# Autodesk Inventor assembly: McCrea_head_walle
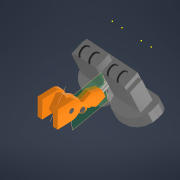
[picture p0: Inventor's stored thumbnail of the model, 180x180]
Saved by Autodesk Inventor 2022 (Build 260153000, 153)
## iProperties
Created: 2022-01-20
Part Number: McCrea_head_walle
Document SubType Name: Assembly
Designer: MatusBarany
Author: MatusBarany
## Documents named in this file (19)
- C:\Users\MatusBarany\Documents\Inventor\wall-e\assembly\McCrea_head_walle.iam
- C:\Users\MatusBarany\Documents\Inventor\wall-e\maxo\McCrea_kabel_walle.ipt
- C:\Users\MatusBarany\Documents\Inventor\wall-e\maxo\McCrea_krk_walle.ipt
- C:\Users\MatusBarany\Documents\Inventor\wall-e\maxo\McCrea_oblucik_walle.ipt
- C:\Users\MatusBarany\Documents\Inventor\wall-e\maxo\McCrea_oko_walle.ipt
- C:\Users\MatusBarany\Documents\Inventor\wall-e\maxo\McCrea_palicka_walle.ipt
- C:\Users\MatusBarany\Documents\Inventor\wall-e\maxo\McCrea_uhco_walle.ipt
- C:\Users\MatusBarany\Documents\Inventor\wall-e\maxo\McCrea_velka_palicka_walle.ipt
- C:\Users\MatusBarany\Documents\Inventor\wall-e\maxo\McCrea_velka_palicka_walle_1.ipt
- C:\Users\MatusBarany\Documents\Inventor\wall-e\maxo\McCrea_velky_krk_walle.ipt
- C:\Users\MatusBarany\Documents\Inventor\wall-e\maxo\McCrea_zadna_cast_oka_walle.ipt
- C:\Users\MatusBarany\Documents\Inventor\wall-e\maxo\McCrea_zadne_oko_walle.ipt
- C:\Users\MatusBarany\Documents\Inventor\wall-e\maxo\McCrea_doska_walle.ipt
- C:\Users\MatusBarany\Documents\Inventor\wall-e\maxo\McCrea_uhco_walle_MIR2.ipt
- C:\Users\MatusBarany\Documents\Inventor\wall-e\maxo\McCrea_zadna_cast_oka_walle_MIR2.ipt
- C:\Users\MatusBarany\Documents\Inventor\wall-e\maxo\McCrea_kabel_walle_MIR.ipt
- C:\Users\MatusBarany\Documents\Inventor\wall-e\maxo\McCrea_oko_walle_MIR2.ipt
- C:\Users\MatusBarany\Documents\Inventor\wall-e\maxo\McCrea_velka_palicka_walle_MIR2.ipt
- C:\Users\MatusBarany\Documents\Inventor\wall-e\maxo\McCrea_zadne_oko_walle_MIR2.ipt
## Components (22 placed, 18 different names)
1. McCrea_krk_walle:1 — Rotational:6, Rotational:8, Insert:2
2. McCrea_oblucik_walle:1 — Rotational:5, Rotational:6, Flush:8
3. McCrea_palicka_walle:1 — Rotational:7
4. McCrea_uhco_walle:1 — Mate:2, Flush:1, Mate:14
5. McCrea_zadna_cast_oka_walle:1 — Rigid:3, Mate:1, Flush:3, Mate:13, Mate:14
6. McCrea_kabel_walle:2 — Mate:3, Mate:15, Mate:16
7. McCrea_oblucik_walle:2 — Rotational:7, Rotational:8, Flush:8
8. McCrea_oko_walle:2 — Rigid:3, Cylindrical:1, Flush:4
9. McCrea_palicka_walle:2 — Rotational:5
10. McCrea_velka_palicka_walle:2 — Cylindrical:1, Flush:4
11. McCrea_velka_palicka_walle_1:2 — Rotational:4, Insert:1
12. McCrea_velky_krk_walle:2 — Insert:1, Flush:2, Insert:2
13. McCrea_zadne_oko_walle:2 — Mate:1, Mate:2, Flush:1, Mate:3, Mate:4, Flush:3, Mate:13, Mate:15, Mate:16, Mate:17, Mate:18, Mate:19, Mate:20, Mate:21
14. McCrea_kabel_walle:3 — Mate:4, Mate:17, Mate:18
15. McCrea_doska_walle:1 — Rotational:4, Mate:19, Mate:20, Mate:21, Flush:9
16. McCrea_uhco_walle_MIR2:1 — Mate:22, Flush:12, Mate:27
17. McCrea_zadna_cast_oka_walle_MIR2:1 — Mate:22, Mate:25, Flush:11, Mate:28, Rigid:4
18. McCrea_kabel_walle_MIR:1 — Mate:23, Mate:24, Mate:26
19. McCrea_oko_walle_MIR2:1 — Flush:10, Rigid:4, Cylindrical:2
20. McCrea_velka_palicka_walle_MIR2:1 — Flush:10, Cylindrical:2
21. McCrea_zadne_oko_walle_MIR2:1 — Mate:23, Mate:24, Mate:25, Flush:11, Mate:26, Flush:12, Mate:27, Mate:28, Mate:29, Mate:30, Mate:31
22. McCrea_kabel_walle_MIR:2 — Mate:29, Mate:30, Mate:31
## Relationships (43: Mate 23, Flush 9, RevoluteJoint 5, WeldJoint 2, Insert 2, CylindricalJoint 2)
- Rigid:3 [WeldJoint]: McCrea_zadna_cast_oka_walle:1 ↔ McCrea_oko_walle:2
- Mate:1: McCrea_zadna_cast_oka_walle:1 ↔ McCrea_zadne_oko_walle:2
- Mate:2: McCrea_uhco_walle:1 ↔ McCrea_zadne_oko_walle:2
- Flush:1: McCrea_uhco_walle:1 ↔ McCrea_zadne_oko_walle:2
- Mate:3: McCrea_kabel_walle:2 ↔ McCrea_zadne_oko_walle:2
- Mate:4: McCrea_zadne_oko_walle:2 ↔ McCrea_kabel_walle:3
- Rotational:4 [RevoluteJoint]: McCrea_velka_palicka_walle_1:2 ↔ McCrea_doska_walle:1
- Insert:1: McCrea_velka_palicka_walle_1:2 ↔ McCrea_velky_krk_walle:2
- Flush:2 (-3.5 mm): McCrea_velky_krk_walle:2
- Flush:3: McCrea_zadna_cast_oka_walle:1 ↔ McCrea_zadne_oko_walle:2
- Cylindrical:1: McCrea_oko_walle:2 ↔ McCrea_velka_palicka_walle:2
- Flush:4: McCrea_oko_walle:2 ↔ McCrea_velka_palicka_walle:2
- Rotational:5 [RevoluteJoint]: McCrea_oblucik_walle:1 ↔ McCrea_palicka_walle:2
- Rotational:6 [RevoluteJoint]: McCrea_krk_walle:1 ↔ McCrea_oblucik_walle:1
- Rotational:7 [RevoluteJoint]: McCrea_palicka_walle:1 ↔ McCrea_oblucik_walle:2
- Rotational:8 [RevoluteJoint]: McCrea_krk_walle:1 ↔ McCrea_oblucik_walle:2
- Flush:8: McCrea_oblucik_walle:1 ↔ McCrea_oblucik_walle:2
- Mate:13: McCrea_zadna_cast_oka_walle:1 ↔ McCrea_zadne_oko_walle:2
- Mate:14: McCrea_uhco_walle:1 ↔ McCrea_zadna_cast_oka_walle:1
- Mate:15: McCrea_kabel_walle:2 ↔ McCrea_zadne_oko_walle:2
- Mate:16: McCrea_kabel_walle:2 ↔ McCrea_zadne_oko_walle:2
- Mate:17: McCrea_zadne_oko_walle:2 ↔ McCrea_kabel_walle:3
- Mate:18: McCrea_zadne_oko_walle:2 ↔ McCrea_kabel_walle:3
- Mate:19: McCrea_zadne_oko_walle:2 ↔ McCrea_doska_walle:1
- Mate:20: McCrea_zadne_oko_walle:2 ↔ McCrea_doska_walle:1
- Mate:21: McCrea_zadne_oko_walle:2 ↔ McCrea_doska_walle:1
- Insert:2: McCrea_krk_walle:1 ↔ McCrea_velky_krk_walle:2
- Flush:9 (-4 mm): McCrea_doska_walle:1
- Mate:22: McCrea_uhco_walle_MIR2:1 ↔ McCrea_zadna_cast_oka_walle_MIR2:1
- Flush:10: McCrea_oko_walle_MIR2:1 ↔ McCrea_velka_palicka_walle_MIR2:1
- Mate:23: McCrea_kabel_walle_MIR:1 ↔ McCrea_zadne_oko_walle_MIR2:1
- Mate:24: McCrea_kabel_walle_MIR:1 ↔ McCrea_zadne_oko_walle_MIR2:1
- Mate:25: McCrea_zadna_cast_oka_walle_MIR2:1 ↔ McCrea_zadne_oko_walle_MIR2:1
- Flush:11: McCrea_zadna_cast_oka_walle_MIR2:1 ↔ McCrea_zadne_oko_walle_MIR2:1
- Mate:26: McCrea_kabel_walle_MIR:1 ↔ McCrea_zadne_oko_walle_MIR2:1
- Flush:12: McCrea_uhco_walle_MIR2:1 ↔ McCrea_zadne_oko_walle_MIR2:1
- Mate:27: McCrea_uhco_walle_MIR2:1 ↔ McCrea_zadne_oko_walle_MIR2:1
- Mate:28: McCrea_zadna_cast_oka_walle_MIR2:1 ↔ McCrea_zadne_oko_walle_MIR2:1
- Mate:29: McCrea_zadne_oko_walle_MIR2:1 ↔ McCrea_kabel_walle_MIR:2
- Mate:30: McCrea_zadne_oko_walle_MIR2:1 ↔ McCrea_kabel_walle_MIR:2
- Mate:31: McCrea_zadne_oko_walle_MIR2:1 ↔ McCrea_kabel_walle_MIR:2
- Rigid:4 [WeldJoint]: McCrea_zadna_cast_oka_walle_MIR2:1 ↔ McCrea_oko_walle_MIR2:1
- Cylindrical:2: McCrea_oko_walle_MIR2:1 ↔ McCrea_velka_palicka_walle_MIR2:1
